# Autodesk Inventor assembly: 組合檔
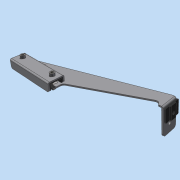
[picture p0: Inventor's stored thumbnail of the model, 180x180]
Saved by Autodesk Inventor 2020 (Build 240168000, 168)
## iProperties
Created: 2015-11-28
Part Number: 組合檔
Document SubType Name: Assembly
Designer: 設計製圖
Author: 設計製圖
## Documents named in this file (11)
- D:\資料庫\設計-3D產品\【May club 】\得利卡-車頂燈架\模型、圖面\old\old ( 草-組合檔 ).iam
- D:\資料庫\設計-3D產品\【May club 】\得利卡-車頂燈架\模型、圖面\old\草-零件 - 複製 (5).ipt
- D:\資料庫\設計-3D產品\【May club 】\得利卡-車頂燈架\模型、圖面\old\草-零件.ipt
- D:\資料庫\設計-3D產品\【May club 】\得利卡-車頂燈架\模型、圖面\old\概-膠條.ipt
- D:\資料庫\設計-3D產品\材料庫\【螺絲】\圓柱內六螺絲\白鐵-圓柱內六螺絲-M8-20.ipt
- D:\資料庫\設計-3D產品\【May club 】\得利卡-車頂燈架\模型、圖面\old\概-泡棉墊(1).ipt
- D:\資料庫\設計-3D產品\【May club 】\得利卡-車頂燈架\模型、圖面\old\概-泡棉墊(2).ipt
- D:\資料庫\設計-3D產品\【May club 】\得利卡-車頂燈架\模型、圖面\old\概-泡棉墊(3).ipt
- D:\資料庫\設計-3D產品\【May club 】\得利卡-車頂燈架\模型、圖面\old\概-膠墊.ipt
- D:\資料庫\設計-3D產品\【May club 】\得利卡-車頂燈架\模型、圖面\old\概-車頂導水槽.ipt
- D:\資料庫\設計-3D產品\【 鐵蹄 】\------鐵蹄工廠素材------ -\焊接螺帽\黑鐵-焊接螺帽-M8.ipt
## Components (13 placed, 10 different names)
1. 概-車頂導水槽:1 — 齊平:9, 齊平:10, 貼合:12, 相切:1, 齊平:13
2. 草-零件 - 複製 (5):1 — 貼合:1, 貼合:2, 齊平:2, 貼合:5, 貼合:6, 貼合:11, 貼合:14, 齊平:11, 齊平:13, 貼合:19, 貼合:20
3. 草-零件:1 — 貼合:7, 齊平:4, 齊平:5, 貼合:8, 齊平:6, 貼合:9, 貼合:10, 齊平:7, 貼合:14, 齊平:11, 貼合:17, 貼合:18
4. 概-膠條:1 — 貼合:1, 貼合:2, 齊平:2, 相切:1
5. 白鐵-圓柱內六螺絲-M8-20:1 — 貼合:16, 齊平:12
6. 白鐵-圓柱內六螺絲-M8-20:2 — 貼合:15, 齊平:12, 貼合:17
7. 黑鐵-焊接螺帽-M8:1 — 貼合:6, 齊平:3, 貼合:16, 貼合:20
8. 黑鐵-焊接螺帽-M8:2 — 貼合:5, 齊平:3, 貼合:15, 貼合:19
9. 概-泡棉墊(1):1 — 貼合:7, 齊平:4, 齊平:5
10. 概-泡棉墊(2):1 — 貼合:8, 齊平:6, 貼合:9, 貼合:13
11. 概-泡棉墊(3):1 — 貼合:10, 齊平:7, 貼合:13
12. 概-膠墊:1 — 貼合:11
13. 白鐵-圓柱內六螺絲-M8-20:3 — 貼合:18
## Relationships (30: Mate 18, Flush 11, Tangent 1)
- 貼合:1 [Mate]: 草-零件 - 複製 (5):1 ↔ 概-膠條:1
- 貼合:2 [Mate]: 草-零件 - 複製 (5):1 ↔ 概-膠條:1
- 齊平:2 [Flush]: 草-零件 - 複製 (5):1 ↔ 概-膠條:1
- 貼合:5 [Mate]: 草-零件 - 複製 (5):1 ↔ 黑鐵-焊接螺帽-M8:2
- 貼合:6 [Mate]: 草-零件 - 複製 (5):1 ↔ 黑鐵-焊接螺帽-M8:1
- 齊平:3 [Flush]: 黑鐵-焊接螺帽-M8:1 ↔ 黑鐵-焊接螺帽-M8:2
- 貼合:7 [Mate]: 草-零件:1 ↔ 概-泡棉墊(1):1
- 齊平:4 [Flush]: 草-零件:1 ↔ 概-泡棉墊(1):1
- 齊平:5 [Flush]: 草-零件:1 ↔ 概-泡棉墊(1):1
- 貼合:8 [Mate]: 草-零件:1 ↔ 概-泡棉墊(2):1
- 齊平:6 [Flush]: 草-零件:1 ↔ 概-泡棉墊(2):1
- 貼合:9 [Mate]: 草-零件:1 ↔ 概-泡棉墊(2):1
- 貼合:10 [Mate]: 草-零件:1 ↔ 概-泡棉墊(3):1
- 齊平:7 [Flush]: 草-零件:1 ↔ 概-泡棉墊(3):1
- 貼合:11 [Mate]: 草-零件 - 複製 (5):1 ↔ 概-膠墊:1
- 齊平:9 [Flush]: 概-車頂導水槽:1
- 齊平:10 [Flush]: 概-車頂導水槽:1
- 貼合:12 [Mate]: 概-車頂導水槽:1
- 貼合:13 [Mate]: 概-泡棉墊(2):1 ↔ 概-泡棉墊(3):1
- 貼合:14 [Mate]: 草-零件 - 複製 (5):1 ↔ 草-零件:1
- 齊平:11 [Flush]: 草-零件 - 複製 (5):1 ↔ 草-零件:1
- 相切:1 [Tangent]: 概-車頂導水槽:1 ↔ 概-膠條:1
- 貼合:15 [Mate]: 白鐵-圓柱內六螺絲-M8-20:2 ↔ 黑鐵-焊接螺帽-M8:2
- 貼合:16 [Mate]: 白鐵-圓柱內六螺絲-M8-20:1 ↔ 黑鐵-焊接螺帽-M8:1
- 齊平:12 [Flush]: 白鐵-圓柱內六螺絲-M8-20:1 ↔ 白鐵-圓柱內六螺絲-M8-20:2
- 齊平:13 [Flush]: 概-車頂導水槽:1 ↔ 草-零件 - 複製 (5):1
- 貼合:17 [Mate]: 草-零件:1 ↔ 白鐵-圓柱內六螺絲-M8-20:2
- 貼合:18 [Mate]: 草-零件:1 ↔ 白鐵-圓柱內六螺絲-M8-20:3
- 貼合:19 [Mate]: 草-零件 - 複製 (5):1 ↔ 黑鐵-焊接螺帽-M8:2
- 貼合:20 [Mate]: 草-零件 - 複製 (5):1 ↔ 黑鐵-焊接螺帽-M8:1
